# Autodesk Inventor assembly: MaleHeader-01
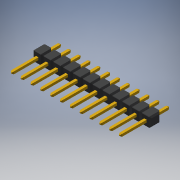
[picture p0: Inventor's stored thumbnail of the model, 180x180]
Saved by Autodesk Inventor 2018 (Build 220112000, 112)
## iProperties
Created: 2017-04-09
Part Number: MaleHeader-01
Document SubType Name: Assembly
Designer: dkt01
Author: dkt01
## Documents named in this file (2)
- C:\Users\dktur\Dropbox\StackLightMonitor\CAD\MaleHeader-01.iam
- C:\Users\dktur\Dropbox\StackLightMonitor\CAD\MaleHeader-01.ipt
## Components (12 placed, 1 different names)
1. MaleHeader-01:1
2. MaleHeader-01:2
3. MaleHeader-01:3
4. MaleHeader-01:4
5. MaleHeader-01:5
6. MaleHeader-01:6
7. MaleHeader-01:7
8. MaleHeader-01:8
9. MaleHeader-01:9
10. MaleHeader-01:10
11. MaleHeader-01:11
12. MaleHeader-01:12
## Component patterns: (12 elements, first: MaleHeader-01:1)
